# Autodesk Inventor assembly: s-assy-unit-j1
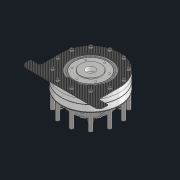
[picture p0: Inventor's stored thumbnail of the model, 180x180]
Saved by Autodesk Inventor 2021 (Build 250183000, 183)
## iProperties
Created: 2021-07-12
Part Number: s-assy-unit-j1
Document SubType Name: Assembly
Designer: yuta0
Mass: 4333.24 g
Surface Area: 5973.62 cm^2
Volume: 1138.09 cm^3
Density: 3.80748 g/cm^3
Author: yuta0
## Documents named in this file (8)
- C:\Users\yuta0\Documents\GitHub\catchrobo_hardware\assy-robot\s-assy-unit-j1.iam
- C:\Users\yuta0\Documents\GitHub\catchrobo_hardware\assy-robot\s-assy-sun_gear.iam
- C:\Users\yuta0\Documents\GitHub\catchrobo_hardware\assy-robot\s-assy-unit-gear.iam
- C:\Users\yuta0\Documents\GitHub\catchrobo_hardware\assy-robot\s-assy-ring_gear-long.iam
- C:\Users\yuta0\Documents\GitHub\catchrobo_hardware\assy-robot\CB4-45.ipt
- C:\Users\yuta0\Documents\GitHub\catchrobo_hardware\assy-robot\carbon_plate1.ipt
- C:\Users\yuta0\Documents\GitHub\catchrobo_hardware\assy-robot\ARF-440E.ipt
- C:\Users\yuta0\Documents\GitHub\catchrobo_hardware\assy-robot\s-assy-unit-j2.iam
## Components (29 placed, 7 different names)
1. s-assy-sun_gear:1 [sub-assembly] — メイト:1, メイト:2
2. s-assy-unit-gear:1 [sub-assembly] — メイト:1, フラッシュ:1, メイト:2, メイト:52, メイト:53
3. s-assy-ring_gear-long:1 [sub-assembly] — メイト:52, メイト:53, メイト:59, メイト:64, メイト:120, メイト:124, フラッシュ:2
4. carbon_plate1:1 — メイト:58, メイト:59, メイト:62, メイト:123
5. s-assy-unit-j2:1 [sub-assembly] — メイト:124, フラッシュ:2
6. unir-spacer5:1 — メイト:63, メイト:64, メイト:120
7. CB4-45:1 — メイト:62, メイト:63
8. unir-spacer5:2
9. CB4-45:2 — メイト:123
10. unir-spacer5:3
11. CB4-45:3
12. unir-spacer5:4
13. CB4-45:4
14. unir-spacer5:5
15. CB4-45:5
16. unir-spacer5:6
17. CB4-45:6
18. unir-spacer5:7
19. CB4-45:7
20. unir-spacer5:8
21. CB4-45:8
22. unir-spacer5:9
23. CB4-45:9
24. unir-spacer5:10
25. CB4-45:10
26. unir-spacer5:11
27. CB4-45:11
28. unir-spacer5:12
29. CB4-45:12
## Component patterns: (12 elements, first: unir-spacer5:1 + CB4-45:1)
## Relationships (14: Mate 12, Flush 2)
- メイト:1 [Mate]: s-assy-sun_gear:1 ↔ s-assy-unit-gear:1
- フラッシュ:1 [Flush]: s-assy-unit-gear:1
- メイト:2 [Mate]: s-assy-sun_gear:1 ↔ s-assy-unit-gear:1
- メイト:52 [Mate]: s-assy-unit-gear:1 ↔ s-assy-ring_gear-long:1
- メイト:53 [Mate]: s-assy-unit-gear:1 ↔ s-assy-ring_gear-long:1
- メイト:58 [Mate]: carbon_plate1:1
- メイト:59 [Mate]: s-assy-ring_gear-long:1 ↔ carbon_plate1:1
- メイト:62 [Mate]: carbon_plate1:1 ↔ CB4-45:1
- メイト:63 [Mate]: unir-spacer5:1 ↔ CB4-45:1
- メイト:64 [Mate]: s-assy-ring_gear-long:1 ↔ unir-spacer5:1
- メイト:120 [Mate]: s-assy-ring_gear-long:1 ↔ unir-spacer5:1
- メイト:123 [Mate]: carbon_plate1:1 ↔ CB4-45:2
- メイト:124 [Mate]: s-assy-ring_gear-long:1 ↔ s-assy-unit-j2:1
- フラッシュ:2 [Flush]: s-assy-ring_gear-long:1 ↔ s-assy-unit-j2:1
